# Autodesk Inventor assembly: 2M2+wzmocnienie
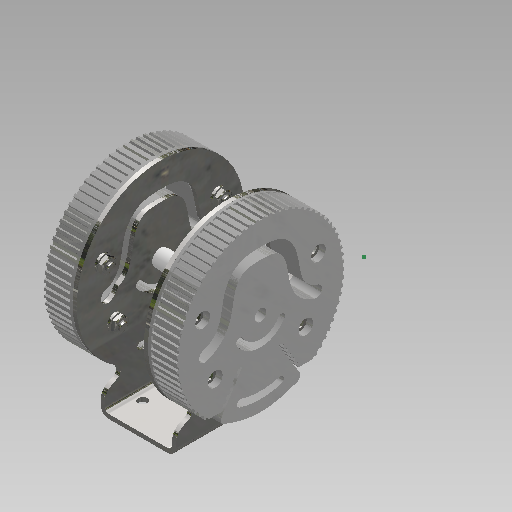
[picture p0: Inventor's stored thumbnail of the model, 512x512]
Saved by Autodesk Inventor 2021 (Build 250183000, 183)
## iProperties
Created: 2021-09-01
Part Number: 2M2+wzmocnienie
Document SubType Name: Assembly
Designer: marci
Mass: 565.352 g
Surface Area: 1657.25 cm^2
Volume: 495.917 cm^3
Density: 1.14001 g/cm^3
Author: marci
## Documents named in this file (8)
- C:\Users\marci\Desktop\Projekt ramienia\2M2\RR-PCSS-2021-2M2.iam
- C:\Users\marci\Desktop\Projekt ramienia\2M2\RR-PCSS-2021-W2M2MA.ipt
- C:\Users\marci\Desktop\Projekt ramienia\2M2\RR-PCSS-2021-2M2.ipt
- C:\Users\marci\Desktop\Projekt ramienia\2M2\RR-PCSS-2021-TŚ.ipt
- C:\Users\marci\Desktop\Projekt ramienia\Nowy folder\pl-PL\ISO 4762(2)\ISO 4762 - M6 x 20ISO.ipt
- C:\Users\marci\Desktop\Projekt ramienia\Nowy folder\pl-PL\ISO 4035(2)\ISO 4035 - M6 - ISO.ipt
- C:\Users\marci\Desktop\Projekt ramienia\Nowy folder\pl-PL\ISO 7089\ISO 7089 - 6 - 140 HV(1).ipt
- C:\Users\marci\Desktop\Projekt ramienia\Nowy folder\pl-PL\DIN EN ISO 7089\DIN EN ISO 7089 -  6.ipt
## Components (28 placed, 7 different names)
1. RR-PCSS-2021-W2M2MA:1 — Wstawiające:1, Wstawiające:2, Równoległe:1, Równoległe:2, Wstawiające:3, Zestawiające:10, Zestawiające:12, Zestawiające:14, Zestawiające:16, Zestawiające:26, Zestawiające:28, Zestawiające:30, Zestawiające:32
2. RR-PCSS-2021-2M2:1 — Wstawiające:2, Równoległe:1, Zestawiające:1, Zestawiające:2, Zestawiające:3, Zestawiające:4, Zestawiające:5, Zestawiające:6, Zestawiające:7, Zestawiające:8, Zestawiające:9, Zestawiające:11, Zestawiające:13, Zestawiające:15
3. RR-PCSS-2021-2M2:2 — Wstawiające:1, Równoległe:2, Zestawiające:17, Zestawiające:18, Zestawiające:19, Zestawiające:20, Zestawiające:21, Zestawiające:22, Zestawiające:23, Zestawiające:24, Zestawiające:25, Zestawiające:27, Zestawiające:29, Zestawiające:31
4. RR-PCSS-2021-TŚ:1 — Wstawiające:3
5. ISO 4762 M6 x 20:1 — Zestawiające:1, Zestawiające:2
6. DIN EN ISO 7089 6:1 — Zestawiające:9, Zestawiające:10, Wstawiające:4
7. ISO 4035 M6:1 — Wstawiające:4
8. ISO 4762 M6 x 20:2 — Zestawiające:3, Zestawiające:4
9. ISO 4762 M6 x 20:3 — Zestawiające:5, Zestawiające:6
10. ISO 4762 M6 x 20:4 — Zestawiające:7, Zestawiające:8
11. DIN EN ISO 7089 6:2 — Zestawiające:11, Zestawiające:12, Wstawiające:5
12. DIN EN ISO 7089 6:3 — Zestawiające:13, Zestawiające:14, Wstawiające:6
13. DIN EN ISO 7089 6:4 — Zestawiające:15, Zestawiające:16, Wstawiające:7
14. ISO 4035 M6:2 — Wstawiające:5
15. ISO 4035 M6:3 — Wstawiające:6
16. ISO 4035 M6:4 — Wstawiające:7
17. ISO 4762 M6 x 20:5 — Zestawiające:17, Zestawiające:18
18. ISO 7089 6:1 — Zestawiające:25, Zestawiające:26, Wstawiające:8
19. ISO 4035 M6:5 — Wstawiające:8
20. ISO 4762 M6 x 20:6 — Zestawiające:19, Zestawiające:20
21. ISO 4762 M6 x 20:7 — Zestawiające:21, Zestawiające:22
22. ISO 4762 M6 x 20:8 — Zestawiające:23, Zestawiające:24
23. ISO 7089 6:2 — Zestawiające:27, Zestawiające:28, Wstawiające:9
24. ISO 7089 6:3 — Zestawiające:29, Zestawiające:30, Wstawiające:10
25. ISO 7089 6:4 — Zestawiające:31, Zestawiające:32, Wstawiające:11
26. ISO 4035 M6:6 — Wstawiające:9
27. ISO 4035 M6:7 — Wstawiające:10
28. ISO 4035 M6:8 — Wstawiające:11
## Relationships (45: Mate 32, Insert 11, Flush 2)
- Wstawiające:1 [Insert]: RR-PCSS-2021-W2M2MA:1 ↔ RR-PCSS-2021-2M2:2
- Wstawiające:2 [Insert]: RR-PCSS-2021-W2M2MA:1 ↔ RR-PCSS-2021-2M2:1
- Równoległe:1 [Flush]: RR-PCSS-2021-W2M2MA:1 ↔ RR-PCSS-2021-2M2:1
- Równoległe:2 [Flush]: RR-PCSS-2021-W2M2MA:1 ↔ RR-PCSS-2021-2M2:2
- Wstawiające:3 [Insert]: RR-PCSS-2021-W2M2MA:1 ↔ RR-PCSS-2021-TŚ:1
- Zestawiające:1 [Mate]: RR-PCSS-2021-2M2:1 ↔ ISO 4762 M6 x 20:1
- Zestawiające:2 [Mate]: RR-PCSS-2021-2M2:1 ↔ ISO 4762 M6 x 20:1
- Zestawiające:3 [Mate]: RR-PCSS-2021-2M2:1 ↔ ISO 4762 M6 x 20:2
- Zestawiające:4 [Mate]: RR-PCSS-2021-2M2:1 ↔ ISO 4762 M6 x 20:2
- Zestawiające:5 [Mate]: RR-PCSS-2021-2M2:1 ↔ ISO 4762 M6 x 20:3
- Zestawiające:6 [Mate]: RR-PCSS-2021-2M2:1 ↔ ISO 4762 M6 x 20:3
- Zestawiające:7 [Mate]: RR-PCSS-2021-2M2:1 ↔ ISO 4762 M6 x 20:4
- Zestawiające:8 [Mate]: RR-PCSS-2021-2M2:1 ↔ ISO 4762 M6 x 20:4
- Zestawiające:9 [Mate]: RR-PCSS-2021-2M2:1 ↔ DIN EN ISO 7089 6:1
- Zestawiające:10 [Mate]: RR-PCSS-2021-W2M2MA:1 ↔ DIN EN ISO 7089 6:1
- Zestawiające:11 [Mate]: RR-PCSS-2021-2M2:1 ↔ DIN EN ISO 7089 6:2
- Zestawiające:12 [Mate]: RR-PCSS-2021-W2M2MA:1 ↔ DIN EN ISO 7089 6:2
- Zestawiające:13 [Mate]: RR-PCSS-2021-2M2:1 ↔ DIN EN ISO 7089 6:3
- Zestawiające:14 [Mate]: RR-PCSS-2021-W2M2MA:1 ↔ DIN EN ISO 7089 6:3
- Zestawiające:15 [Mate]: RR-PCSS-2021-2M2:1 ↔ DIN EN ISO 7089 6:4
- Zestawiające:16 [Mate]: RR-PCSS-2021-W2M2MA:1 ↔ DIN EN ISO 7089 6:4
- Wstawiające:4 [Insert]: DIN EN ISO 7089 6:1 ↔ ISO 4035 M6:1
- Wstawiające:5 [Insert]: DIN EN ISO 7089 6:2 ↔ ISO 4035 M6:2
- Wstawiające:6 [Insert]: DIN EN ISO 7089 6:3 ↔ ISO 4035 M6:3
- Wstawiające:7 [Insert]: DIN EN ISO 7089 6:4 ↔ ISO 4035 M6:4
- Zestawiające:17 [Mate]: RR-PCSS-2021-2M2:2 ↔ ISO 4762 M6 x 20:5
- Zestawiające:18 [Mate]: RR-PCSS-2021-2M2:2 ↔ ISO 4762 M6 x 20:5
- Zestawiające:19 [Mate]: RR-PCSS-2021-2M2:2 ↔ ISO 4762 M6 x 20:6
- Zestawiające:20 [Mate]: RR-PCSS-2021-2M2:2 ↔ ISO 4762 M6 x 20:6
- Zestawiające:21 [Mate]: RR-PCSS-2021-2M2:2 ↔ ISO 4762 M6 x 20:7
- Zestawiające:22 [Mate]: RR-PCSS-2021-2M2:2 ↔ ISO 4762 M6 x 20:7
- Zestawiające:23 [Mate]: RR-PCSS-2021-2M2:2 ↔ ISO 4762 M6 x 20:8
- Zestawiające:24 [Mate]: RR-PCSS-2021-2M2:2 ↔ ISO 4762 M6 x 20:8
- Zestawiające:25 [Mate]: RR-PCSS-2021-2M2:2 ↔ ISO 7089 6:1
- Zestawiające:26 [Mate]: RR-PCSS-2021-W2M2MA:1 ↔ ISO 7089 6:1
- Zestawiające:27 [Mate]: RR-PCSS-2021-2M2:2 ↔ ISO 7089 6:2
- Zestawiające:28 [Mate]: RR-PCSS-2021-W2M2MA:1 ↔ ISO 7089 6:2
- Zestawiające:29 [Mate]: RR-PCSS-2021-2M2:2 ↔ ISO 7089 6:3
- Zestawiające:30 [Mate]: RR-PCSS-2021-W2M2MA:1 ↔ ISO 7089 6:3
- Zestawiające:31 [Mate]: RR-PCSS-2021-2M2:2 ↔ ISO 7089 6:4
- Zestawiające:32 [Mate]: RR-PCSS-2021-W2M2MA:1 ↔ ISO 7089 6:4
- Wstawiające:8 [Insert]: ISO 7089 6:1 ↔ ISO 4035 M6:5
- Wstawiające:9 [Insert]: ISO 7089 6:2 ↔ ISO 4035 M6:6
- Wstawiające:10 [Insert]: ISO 7089 6:3 ↔ ISO 4035 M6:7
- Wstawiające:11 [Insert]: ISO 7089 6:4 ↔ ISO 4035 M6:8
